# Autodesk Inventor assembly: LeftFootUnit
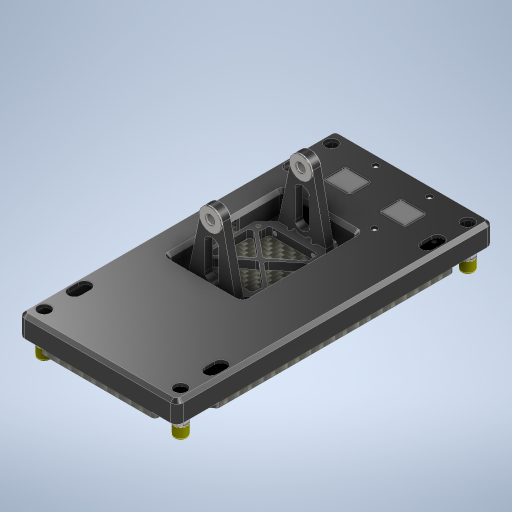
[picture p0: Inventor's stored thumbnail of the model, 512x512]
Saved by Autodesk Inventor 2024.2 (Build 282272000, 272)
## iProperties
Created: 2024-01-07
Part Number: LeftFootUnit
Document SubType Name: Assembly
Designer: Masato Kubotera
Mass: 227.586 g
Surface Area: 1232.19 cm^2
Volume: 155.4 cm^3
Density: 1.46452 g/cm^3
Author: Masato Kubotera
## Documents named in this file (16)
- C:\Users\masato\OneDrive - Chiba Institute of Technology\CIT Brains\RoboCup2024\SUSTAINA-OP2-DEV\NativeFiles\Boby\LowerLimb\Feet\LeftFootUnit.iam
- C:\Users\masato\OneDrive - Chiba Institute of Technology\CIT Brains\RoboCup2024\SUSTAINA-OP2-DEV\NativeFiles\Boby\LowerLimb\LegRollSliderFrame.ipt
- C:\Users\masato\OneDrive - Chiba Institute of Technology\CIT Brains\RoboCup2024\SUSTAINA-OP2-DEV\NativeFiles\Boby\COTS\Bushes\GFM-0608-06.ipt
- C:\Users\masato\OneDrive - Chiba Institute of Technology\CIT Brains\RoboCup2024\SUSTAINA-OP2-DEV\NativeFiles\Boby\COTS\Washers\Metal\UUW-0614-05H.ipt
- C:\Users\masato\OneDrive - Chiba Institute of Technology\CIT Brains\RoboCup2024\SUSTAINA-OP2-DEV\NativeFiles\Boby\COTS\Screws\CapScrew\UC-0310.ipt
- C:\Users\masato\OneDrive - Chiba Institute of Technology\CIT Brains\RoboCup2024\SUSTAINA-OP2-DEV\NativeFiles\Boby\LowerLimb\Feet\FootBraceFrame.ipt
- C:\Users\masato\OneDrive - Chiba Institute of Technology\CIT Brains\RoboCup2024\SUSTAINA-OP2-DEV\NativeFiles\Boby\LowerLimb\Feet\FootSoleFrame.ipt
- C:\Users\masato\OneDrive - Chiba Institute of Technology\CIT Brains\RoboCup2024\SUSTAINA-OP2-DEV\NativeFiles\Boby\COTS\Screws\CapScrew\UC-0308.ipt
- C:\Users\masato\OneDrive - Chiba Institute of Technology\CIT Brains\RoboCup2024\SUSTAINA-OP2-DEV\NativeFiles\Boby\COTS\MisumiComponents\URLM8\URLM8.iam
- C:\Users\masato\OneDrive - Chiba Institute of Technology\CIT Brains\RoboCup2024\SUSTAINA-OP2-DEV\NativeFiles\Boby\COTS\ElectronicComponents\SC700-40kg.ipt
- C:\Users\masato\OneDrive - Chiba Institute of Technology\CIT Brains\RoboCup2024\SUSTAINA-OP2-DEV\NativeFiles\Boby\COTS\Screws\CapScrew\UC-0306.ipt
- C:\Users\masato\OneDrive - Chiba Institute of Technology\CIT Brains\RoboCup2024\SUSTAINA-OP2-DEV\NativeFiles\Boby\LowerLimb\Feet\LeftFootCover.ipt
- C:\Users\masato\OneDrive - Chiba Institute of Technology\CIT Brains\RoboCup2024\SUSTAINA-OP2-DEV\NativeFiles\Boby\COTS\Washers\Resin\TT-0614-05.ipt
- C:\Users\masato\OneDrive - Chiba Institute of Technology\CIT Brains\RoboCup2024\SUSTAINA-OP2-DEV\NativeFiles\Boby\COTS\Spacers\WBN-305.ipt
- C:\Users\masato\OneDrive - Chiba Institute of Technology\CIT Brains\RoboCup2024\SUSTAINA-OP2-DEV\NativeFiles\Boby\CustomPCBs\SUSTAINA-STRAINGAUGE-SENSING-BOARD.ipt
- C:\Users\masato\OneDrive - Chiba Institute of Technology\CIT Brains\RoboCup2024\SUSTAINA-OP2-DEV\NativeFiles\Boby\COTS\Nuts\UNT-03.ipt
## Components (56 placed, 15 different names)
1. LegRollSliderFrame:1 — Mate:1, Angle:1, Flush:2, Flush:3, Insert:1, Insert:3, Insert:7, Insert:8, Insert:11, Insert:12, Mate:2
2. LegRollSliderFrame:2 — Flush:2, Flush:3, Insert:2, Insert:4, Insert:9, Insert:10, Insert:13, Insert:14
3. FootBraceFrame:1 — Insert:11, Insert:12, Insert:13, Insert:14, Insert:15, Insert:16, Insert:17, Insert:18
4. FootSoleFrame:1 — Insert:15, Insert:16, Insert:18, Insert:19, Insert:20, Insert:21, Insert:22, Insert:23, Insert:24, Insert:25, Insert:26, Insert:27, Insert:28, Insert:29, Insert:30, Flush:4, Flush:5, Flush:6, Insert:53, Insert:54, Insert:55, Insert:56, Insert:57, Insert:58, Insert:59, Insert:60, Insert:61, Insert:62, Insert:63, Insert:64, Insert:65, Insert:66, Insert:67, Insert:68, Insert:17
5. SUSTAINA-STRAINGAUGE-SENSING-BOARD:1 — Insert:49, Insert:50, Insert:51, Insert:52
6. LeftFootCover:1 — Flush:4, Flush:5, Flush:6
7. GFM-0608-06:1 — Insert:1
8. GFM-0608-06:2 — Insert:2
9. SC700-40kg:1 — Insert:23, Insert:24, Insert:31, Insert:35, Insert:41, Insert:45
10. SC700-40kg:2 — Insert:25, Insert:26, Insert:32, Insert:36, Insert:42, Insert:46
11. SC700-40kg:3 — Insert:27, Insert:28, Insert:33, Insert:37, Insert:47, Insert:43
12. SC700-40kg:4 — Insert:29, Insert:30, Insert:34, Insert:38, Insert:48, Insert:44
13. UC-0306:1 — Insert:35
14. UC-0306:2 — Insert:36
15. UC-0306:3 — Insert:37
16. UC-0306:4 — Insert:38
17. UC-0308:9 — Insert:41
18. UC-0308:10 — Insert:42
19. UC-0308:12 — Insert:43
20. UC-0308:11 — Insert:44
21. UC-0308:5 — Insert:45
22. UC-0308:6 — Insert:46
23. UC-0308:7 — Insert:47
24. UC-0308:8 — Insert:48
25. UC-0310:1 — Insert:7
26. UC-0310:2 — Insert:8
27. UC-0310:3 — Insert:9
28. UC-0310:4 — Insert:10
29. UC-0308:1 — Insert:19
30. UC-0308:2 — Insert:20
31. UC-0308:3 — Insert:21
32. UC-0308:4 — Insert:22
33. WBN-305:4 — Insert:51, Angle:2, Insert:56
34. WBN-305:1 — Insert:50, Angle:3, Insert:53
35. WBN-305:2 — Insert:52, Angle:4, Insert:55
36. WBN-305:3 — Insert:49, Angle:5, Insert:54
37. URLM8:1 [sub-assembly] — Insert:31, Angle:6
38. URLM8:2 [sub-assembly] — Insert:32, Angle:7
39. URLM8:3 [sub-assembly] — Insert:33, Angle:8
40. URLM8:4 [sub-assembly] — Insert:34, Angle:9
41. TT-0614-05:2 — Insert:3, Insert:5
42. TT-0614-05:1 — Insert:4, Insert:6
43. UUW-0614-05H:1 — Insert:5
44. UUW-0614-05H:2 — Insert:6
45. UNT-03:1 — Insert:57
46. UNT-03:2 — Insert:58
47. UNT-03:3 — Insert:61
48. UNT-03:4 — Insert:62
49. UNT-03:5 — Insert:59
50. UNT-03:6 — Insert:60
51. UNT-03:7 — Insert:63
52. UNT-03:8 — Insert:64
53. UNT-03:9 — Insert:67
54. UNT-03:10 — Insert:68
55. UNT-03:11 — Insert:65
56. UNT-03:12 — Insert:66
## Relationships (82: Insert 66, Angle 9, Flush 5, Mate 2)
- Mate:1: LegRollSliderFrame:1
- Angle:1 (180 deg): LegRollSliderFrame:1
- Flush:2: LegRollSliderFrame:1 ↔ LegRollSliderFrame:2
- Flush:3: LegRollSliderFrame:1 ↔ LegRollSliderFrame:2
- Insert:1: LegRollSliderFrame:1 ↔ GFM-0608-06:1
- Insert:2: LegRollSliderFrame:2 ↔ GFM-0608-06:2
- Insert:3: LegRollSliderFrame:1 ↔ TT-0614-05:2
- Insert:4: LegRollSliderFrame:2 ↔ TT-0614-05:1
- Insert:5: TT-0614-05:2 ↔ UUW-0614-05H:1
- Insert:6: TT-0614-05:1 ↔ UUW-0614-05H:2
- Insert:7: LegRollSliderFrame:1 ↔ UC-0310:1
- Insert:8: LegRollSliderFrame:1 ↔ UC-0310:2
- Insert:9: LegRollSliderFrame:2 ↔ UC-0310:3
- Insert:10: LegRollSliderFrame:2 ↔ UC-0310:4
- Insert:11: LegRollSliderFrame:1 ↔ FootBraceFrame:1
- Insert:12: LegRollSliderFrame:1 ↔ FootBraceFrame:1
- Insert:13: LegRollSliderFrame:2 ↔ FootBraceFrame:1
- Insert:14: LegRollSliderFrame:2 ↔ FootBraceFrame:1
- Mate:2 (16 mm): LegRollSliderFrame:1
- Insert:15: FootBraceFrame:1 ↔ FootSoleFrame:1
- Insert:16: FootBraceFrame:1 ↔ FootSoleFrame:1
- Insert:17: FootBraceFrame:1 ↔ FootSoleFrame:1
- Insert:18: FootBraceFrame:1 ↔ FootSoleFrame:1
- Insert:19: FootSoleFrame:1 ↔ UC-0308:1
- Insert:20: FootSoleFrame:1 ↔ UC-0308:2
- Insert:21: FootSoleFrame:1 ↔ UC-0308:3
- Insert:22: FootSoleFrame:1 ↔ UC-0308:4
- Insert:23: FootSoleFrame:1 ↔ SC700-40kg:1
- Insert:24: FootSoleFrame:1 ↔ SC700-40kg:1
- Insert:25: FootSoleFrame:1 ↔ SC700-40kg:2
- Insert:26: FootSoleFrame:1 ↔ SC700-40kg:2
- Insert:27: FootSoleFrame:1 ↔ SC700-40kg:3
- Insert:28: FootSoleFrame:1 ↔ SC700-40kg:3
- Insert:29: FootSoleFrame:1 ↔ SC700-40kg:4
- Insert:30: FootSoleFrame:1 ↔ SC700-40kg:4
- Insert:31: SC700-40kg:1 ↔ URLM8:1
- Insert:32: SC700-40kg:2 ↔ URLM8:2
- Insert:33: SC700-40kg:3 ↔ URLM8:3
- Insert:34: SC700-40kg:4 ↔ URLM8:4
- Insert:35: SC700-40kg:1 ↔ UC-0306:1
- Insert:36: SC700-40kg:2 ↔ UC-0306:2
- Insert:37: SC700-40kg:3 ↔ UC-0306:3
- Insert:38: SC700-40kg:4 ↔ UC-0306:4
- Flush:4: FootSoleFrame:1 ↔ LeftFootCover:1
- Flush:5: FootSoleFrame:1 ↔ LeftFootCover:1
- Flush:6: FootSoleFrame:1 ↔ LeftFootCover:1
- Insert:41: SC700-40kg:1 ↔ UC-0308:9
- Insert:42: SC700-40kg:2 ↔ UC-0308:10
- Insert:43: SC700-40kg:3 ↔ UC-0308:12
- Insert:44: SC700-40kg:4 ↔ UC-0308:11
- Insert:45: SC700-40kg:1 ↔ UC-0308:5
- Insert:46: SC700-40kg:2 ↔ UC-0308:6
- Insert:47: SC700-40kg:3 ↔ UC-0308:7
- Insert:48: SC700-40kg:4 ↔ UC-0308:8
- Insert:49: SUSTAINA-STRAINGAUGE-SENSING-BOARD:1 ↔ WBN-305:3
- Insert:50: SUSTAINA-STRAINGAUGE-SENSING-BOARD:1 ↔ WBN-305:1
- Insert:51: SUSTAINA-STRAINGAUGE-SENSING-BOARD:1 ↔ WBN-305:4
- Insert:52: SUSTAINA-STRAINGAUGE-SENSING-BOARD:1 ↔ WBN-305:2
- Angle:2 (0 deg): WBN-305:4
- Angle:3 (0 deg): WBN-305:1
- Angle:4 (0 deg): WBN-305:2
- Angle:5 (0 deg): WBN-305:3
- Insert:53: FootSoleFrame:1 ↔ WBN-305:1
- Insert:54: FootSoleFrame:1 ↔ WBN-305:3
- Insert:55: FootSoleFrame:1 ↔ WBN-305:2
- Insert:56: FootSoleFrame:1 ↔ WBN-305:4
- Insert:57: FootSoleFrame:1 ↔ UNT-03:1
- Insert:58: FootSoleFrame:1 ↔ UNT-03:2
- Insert:59: FootSoleFrame:1 ↔ UNT-03:5
- Insert:60: FootSoleFrame:1 ↔ UNT-03:6
- Insert:61: FootSoleFrame:1 ↔ UNT-03:3
- Insert:62: FootSoleFrame:1 ↔ UNT-03:4
- Insert:63: FootSoleFrame:1 ↔ UNT-03:7
- Insert:64: FootSoleFrame:1 ↔ UNT-03:8
- Insert:65: FootSoleFrame:1 ↔ UNT-03:11
- Insert:66: FootSoleFrame:1 ↔ UNT-03:12
- Insert:67: FootSoleFrame:1 ↔ UNT-03:9
- Insert:68: FootSoleFrame:1 ↔ UNT-03:10
- Angle:6 (0 deg): URLM8:1
- Angle:7 (0 deg): URLM8:2
- Angle:8 (0 deg): URLM8:3
- Angle:9 (0 deg): URLM8:4
